# Autodesk Inventor assembly: motorWithBlades
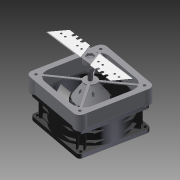
[picture p0: Inventor's stored thumbnail of the model, 180x180]
Saved by Autodesk Inventor 2014 SP2 (Build 180246200, 246)
## iProperties
Created: 2020-05-30
Part Number: motorWithBlades
Document SubType Name: Assembly
Designer: GauchoHP
Author: GauchoHP
## Documents named in this file (8)
- E:\Dati\Documenti_Emanuele\Svago - Varie\tosaerba\LAWNMOWER-ROBOT-from-Hoverboard-\LawnmowerMechanicalProject\3D PROJECT - INVENTOR 2014\motor with blades\motorWithBlades.iam
- E:\Dati\Documenti_Emanuele\Svago - Varie\tosaerba\LAWNMOWER-ROBOT-from-Hoverboard-\LawnmowerMechanicalProject\3D PROJECT - INVENTOR 2014\motor with blades\motorSupportSpacer.ipt
- E:\Dati\Documenti_Emanuele\Svago - Varie\tosaerba\LAWNMOWER-ROBOT-from-Hoverboard-\LawnmowerMechanicalProject\3D PROJECT - INVENTOR 2014\motor with blades\Imported Components\motor\motor.iam
- E:\Dati\Documenti_Emanuele\Svago - Varie\tosaerba\LAWNMOWER-ROBOT-from-Hoverboard-\LawnmowerMechanicalProject\3D PROJECT - INVENTOR 2014\motor with blades\motorSupportShaft.ipt
- C:\Users\GauchoHP\Documents\Inventor\Content Center Files\R2014\en-US\JIS B 1180  A+B\JIS B 1180 - A + B M5x40x6,88 - 10.ipt
- E:\Dati\Documenti_Emanuele\Svago - Varie\tosaerba\LAWNMOWER-ROBOT-from-Hoverboard-\LawnmowerMechanicalProject\3D PROJECT - INVENTOR 2014\motor with blades\blade.ipt
- E:\Dati\Documenti_Emanuele\Svago - Varie\tosaerba\LAWNMOWER-ROBOT-from-Hoverboard-\LawnmowerMechanicalProject\3D PROJECT - INVENTOR 2014\motor with blades\support_for_2_blades.ipt
- C:\Users\GauchoHP\Documents\Inventor\Content Center Files\R2014\en-US\ANSI B 18.2.4.1 M(1)\ANSI B 18.2.4.1 M - M5 x 0,8Style 1.ipt
## Components (9 placed, 7 different names)
1. motorSupportSpacer:1 — Mate:1, Mate:7, Mate:8
2. motor:1 [sub-assembly] — Mate:1, Mate:2, Mate:5, Mate:6, Mate:8
3. motorSupportShaft:1 — Mate:2, Mate:3, Mate:4, Mate:5, Mate:6, Mate:7
4. JIS B 1180 A+B - Metric A + B M5x40:1 — Mate:3, Mate:4, Mate:10, Flush:1, Mate:11, Mate:13
5. blade:1 — Mate:15, Mate:16, Mate:17
6. support_for_2_blades:1 — Mate:11, Mate:12, Mate:14, Mate:15, Mate:16, Mate:17, Mate:18, Mate:19, Mate:20
7. Hex Nut Metric M5 x 0,8:1 — Mate:10, Flush:1, Mate:12
8. Hex Nut Metric M5 x 0,8:2 — Mate:13, Mate:14
9. blade:2 — Mate:18, Mate:19, Mate:20
## Relationships (20: Mate 19, Flush 1)
- Mate:1: motorSupportSpacer:1 ↔ motor:1
- Mate:2: motor:1 ↔ motorSupportShaft:1
- Mate:3 (0.508 mm): motorSupportShaft:1 ↔ JIS B 1180 A+B - Metric A + B M5x40:1
- Mate:4: motorSupportShaft:1 ↔ JIS B 1180 A+B - Metric A + B M5x40:1
- Mate:5: motor:1 ↔ motorSupportShaft:1
- Mate:6: motor:1 ↔ motorSupportShaft:1
- Mate:7: motorSupportSpacer:1 ↔ motorSupportShaft:1
- Mate:8 (0.508 mm): motorSupportSpacer:1 ↔ motor:1
- Mate:10: JIS B 1180 A+B - Metric A + B M5x40:1 ↔ Hex Nut Metric M5 x 0,8:1
- Flush:1: JIS B 1180 A+B - Metric A + B M5x40:1 ↔ Hex Nut Metric M5 x 0,8:1
- Mate:11: JIS B 1180 A+B - Metric A + B M5x40:1 ↔ support_for_2_blades:1
- Mate:12: support_for_2_blades:1 ↔ Hex Nut Metric M5 x 0,8:1
- Mate:13: JIS B 1180 A+B - Metric A + B M5x40:1 ↔ Hex Nut Metric M5 x 0,8:2
- Mate:14: support_for_2_blades:1 ↔ Hex Nut Metric M5 x 0,8:2
- Mate:15: blade:1 ↔ support_for_2_blades:1
- Mate:16: blade:1 ↔ support_for_2_blades:1
- Mate:17: blade:1 ↔ support_for_2_blades:1
- Mate:18: support_for_2_blades:1 ↔ blade:2
- Mate:19: support_for_2_blades:1 ↔ blade:2
- Mate:20: support_for_2_blades:1 ↔ blade:2
